# Autodesk Inventor assembly: Hand
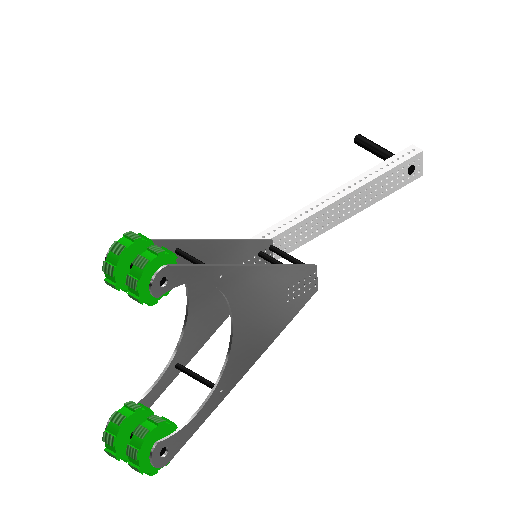
[picture p0: Inventor's stored thumbnail of the model, 512x512]
Saved by Autodesk Inventor 2025.3 (Build 293356000, 356)
## iProperties
Created: 2026-05-13
Part Number: Hand
Document SubType Name: Assembly
Designer: djair.oliveira
Author: djair.oliveira
## Documents named in this file (7)
- C:\Users\djair.oliveira\Documents\GitHub\MT_2026\CAD\Model A\Hand\Hand.iam
- C:\Users\djair.oliveira\Documents\GitHub\MT_2026\CAD\Model A\Hand\Forja - Base1 Hand.ipt
- C:\Users\djair.oliveira\Documents\GitHub\MT_2026\CAD\Model A\Hand\Articulation Hand.ipt
- C:\Users\djair.oliveira\Documents\GitHub\MT_2026\CAD\Model A\Hand\Chapa Base - Hand.ipt
- C:\Users\djair.oliveira\Documents\GitHub\MT_2026\CAD\Model A\Hand\Coletor - Hand.ipt
- C:\Users\djair.oliveira\Documents\GitHub\MT_2026\CAD\Model A\Hand\Suporte - Chapa Base Hand.ipt
- C:\Users\djair.oliveira\Documents\GitHub\MT_2026\CAD\Model A\Hand\Suporte - Chapa Base Hand_MIR.ipt
## Components (12 placed, 6 different names)
1. Forja - Base1 Hand:1 — Alinhado:1, Coincidente:1, Coincidente:2, Coincidente:3, Coincidente:4, Alinhado:2
2. Articulation Hand:1 — Alinhado:1, Coincidente:1, Coincidente:25, Coincidente:26, Coincidente:27
3. Chapa Base - Hand:1 — Coincidente:2, Coincidente:3, Coincidente:4, Coincidente:12, Coincidente:13, Coincidente:14, Coincidente:15, Coincidente:16, Coincidente:18, Coincidente:19, Coincidente:20, Coincidente:21, Coincidente:22, Coincidente:28, Coincidente:31
4. Chapa Base - Hand:2 — Coincidente:23, Coincidente:24, Coincidente:29, Coincidente:30, Coincidente:32, Coincidente:33, Coincidente:34
5. Suporte - Chapa Base Hand:1 — Coincidente:13, Coincidente:21, Coincidente:32
6. Suporte - Chapa Base Hand:2 — Coincidente:15, Coincidente:18, Coincidente:34
7. Suporte - Chapa Base Hand:3 — Coincidente:16, Coincidente:22
8. Suporte - Chapa Base Hand:5 — Coincidente:14, Coincidente:20, Coincidente:33
9. Suporte - Chapa Base Hand:6 — Coincidente:12, Coincidente:19
10. Suporte - Chapa Base Hand_MIR:1 — Coincidente:23, Coincidente:24
11. Coletor - Hand:1 — Coincidente:30, Coincidente:31
12. Coletor - Hand:2 — Coincidente:28, Coincidente:29
## Relationships (28: Mate 26, Flush 2)
- Alinhado:1 [Flush]: Forja - Base1 Hand:1 ↔ Articulation Hand:1
- Coincidente:1 [Mate]: Forja - Base1 Hand:1 ↔ Articulation Hand:1
- Coincidente:2 [Mate]: Forja - Base1 Hand:1 ↔ Chapa Base - Hand:1
- Coincidente:3 [Mate]: Forja - Base1 Hand:1 ↔ Chapa Base - Hand:1
- Coincidente:4 [Mate]: Forja - Base1 Hand:1 ↔ Chapa Base - Hand:1
- Coincidente:12 [Mate]: Chapa Base - Hand:1 ↔ Suporte - Chapa Base Hand:6
- Coincidente:13 [Mate]: Chapa Base - Hand:1 ↔ Suporte - Chapa Base Hand:1
- Coincidente:14 [Mate]: Chapa Base - Hand:1 ↔ Suporte - Chapa Base Hand:5
- Coincidente:15 [Mate]: Chapa Base - Hand:1 ↔ Suporte - Chapa Base Hand:2
- Coincidente:16 [Mate]: Chapa Base - Hand:1 ↔ Suporte - Chapa Base Hand:3
- Coincidente:18 [Mate]: Chapa Base - Hand:1 ↔ Suporte - Chapa Base Hand:2
- Coincidente:19 [Mate]: Chapa Base - Hand:1 ↔ Suporte - Chapa Base Hand:6
- Coincidente:20 [Mate]: Chapa Base - Hand:1 ↔ Suporte - Chapa Base Hand:5
- Coincidente:21 [Mate]: Chapa Base - Hand:1 ↔ Suporte - Chapa Base Hand:1
- Alinhado:2 [Flush] (-25.4 mm): Forja - Base1 Hand:1
- Coincidente:22 [Mate]: Chapa Base - Hand:1 ↔ Suporte - Chapa Base Hand:3
- Coincidente:23 [Mate]: Chapa Base - Hand:2 ↔ Suporte - Chapa Base Hand_MIR:1
- Coincidente:24 [Mate]: Chapa Base - Hand:2 ↔ Suporte - Chapa Base Hand_MIR:1
- Coincidente:25 [Mate]: Articulation Hand:1
- Coincidente:26 [Mate] (-50.8 mm): Articulation Hand:1
- Coincidente:27 [Mate]: Articulation Hand:1
- Coincidente:28 [Mate]: Chapa Base - Hand:1 ↔ Coletor - Hand:2
- Coincidente:29 [Mate]: Chapa Base - Hand:2 ↔ Coletor - Hand:2
- Coincidente:30 [Mate]: Chapa Base - Hand:2 ↔ Coletor - Hand:1
- Coincidente:31 [Mate]: Chapa Base - Hand:1 ↔ Coletor - Hand:1
- Coincidente:32 [Mate]: Chapa Base - Hand:2 ↔ Suporte - Chapa Base Hand:1
- Coincidente:33 [Mate]: Chapa Base - Hand:2 ↔ Suporte - Chapa Base Hand:5
- Coincidente:34 [Mate]: Chapa Base - Hand:2 ↔ Suporte - Chapa Base Hand:2
